# Autodesk Inventor assembly: sample-transfer
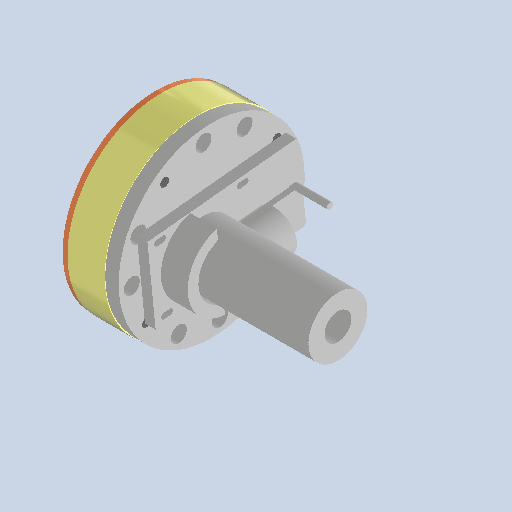
[picture p0: Inventor's stored thumbnail of the model, 512x512]
Saved by Autodesk Inventor 2026.1 (Build 301233000, 233)
## iProperties
Created: 2019-08-16
Part Number: sample-transfer
Document SubType Name: Assembly
Designer: rainer
Author: rainer
## Documents named in this file (9)
- C:\Users\user\Desktop\setup_inventor_2025\single-objective\sample-transfer.iam
- C:\Users\user\Desktop\setup_inventor_2025\single-objective\sample-transfer_plate.ipt
- C:\Users\user\Desktop\setup_inventor_2025\single-objective\sample-transfer_rod.ipt
- C:\Users\user\Desktop\setup_inventor_2025\single-objective\sample-transfer_insulation.ipt
- C:\Users\user\Desktop\setup_inventor_2025\single-objective\sample-transfer_adapter-plate.ipt
- C:\Users\user\Desktop\setup_inventor_2025\single-objective\sample-transfer_insulation-disk.ipt
- C:\Users\user\Desktop\setup_inventor_2025\single-objective\sample-transfer_slider-plate.ipt
- C:\Users\user\Desktop\setup_inventor_2025\single-objective\sample-transfer_shuttle-mockup.ipt
- C:\Users\user\Desktop\setup_inventor_2025\single-objective\sample-transfer_slider.ipt
## Components (8 placed, 8 different names)
1. sample-transfer_plate:1 — Mate:1, Mate:2, Mate:3, Mate:4, Mate:5, Mate:6
2. sample-transfer_rod:1 — Mate:1, Mate:2, Mate:3, Mate:10
3. sample-transfer_insulation:1 — Mate:4, Mate:5, Mate:6, Mate:7, Mate:8, Mate:9, Mate:19
4. sample-transfer_adapter-plate:1 — Mate:7, Mate:8, Mate:11, Mate:12, Mate:13, Mate:19
5. sample-transfer_insulation-disk:1 — Mate:9, Mate:10, Mate:15
6. sample-transfer_slider-plate:1 — Mate:11, Mate:12, Mate:13, Mate:14, Mate:16, Mate:18, Angle:1
7. sample-transfer_shuttle-mockup:1 — Mate:14, Mate:15, Angle:1
8. sample-transfer_slider:1 — Mate:16, Mate:18
## Relationships (19: Mate 18, Angle 1)
- Mate:1: sample-transfer_plate:1 ↔ sample-transfer_rod:1
- Mate:2: sample-transfer_plate:1 ↔ sample-transfer_rod:1
- Mate:3: sample-transfer_plate:1 ↔ sample-transfer_rod:1
- Mate:4: sample-transfer_plate:1 ↔ sample-transfer_insulation:1
- Mate:5: sample-transfer_plate:1 ↔ sample-transfer_insulation:1
- Mate:6: sample-transfer_plate:1 ↔ sample-transfer_insulation:1
- Mate:7: sample-transfer_insulation:1 ↔ sample-transfer_adapter-plate:1
- Mate:8: sample-transfer_insulation:1 ↔ sample-transfer_adapter-plate:1
- Mate:9: sample-transfer_insulation:1 ↔ sample-transfer_insulation-disk:1
- Mate:10: sample-transfer_rod:1 ↔ sample-transfer_insulation-disk:1
- Mate:11: sample-transfer_adapter-plate:1 ↔ sample-transfer_slider-plate:1
- Mate:12: sample-transfer_adapter-plate:1 ↔ sample-transfer_slider-plate:1
- Mate:13: sample-transfer_adapter-plate:1 ↔ sample-transfer_slider-plate:1
- Mate:14: sample-transfer_slider-plate:1 ↔ sample-transfer_shuttle-mockup:1
- Mate:15: sample-transfer_insulation-disk:1 ↔ sample-transfer_shuttle-mockup:1
- Mate:16: sample-transfer_slider-plate:1 ↔ sample-transfer_slider:1
- Mate:18: sample-transfer_slider-plate:1 ↔ sample-transfer_slider:1
- Mate:19: sample-transfer_insulation:1 ↔ sample-transfer_adapter-plate:1
- Angle:1 (0 deg): sample-transfer_slider-plate:1 ↔ sample-transfer_shuttle-mockup:1
